# Autodesk Inventor assembly: am 42 Tooth Pulley Full
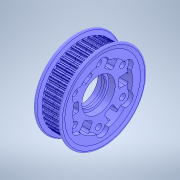
[picture p0: Inventor's stored thumbnail of the model, 180x180]
Saved by Autodesk Inventor 2021 (Build 250183000, 183)
## iProperties
Created: 2021-02-24
Part Number: am 42 Tooth Pulley Full
Document SubType Name: Assembly
Designer: aidan
Author: aidan
## Documents named in this file (2)
- C:\Users\aidan\Desktop\T3 Robotics\CAD\Generic and Stock\am 42 Tooth Pulley Full.iam
- C:\Users\aidan\Desktop\T3 Robotics\CAD\Generic and Stock\am 42 Tooth Pulley half.ipt
## Components (2 placed, 1 different names)
1. am 42 Tooth Pulley half:1 — Mate:2, Mate:3, Mate:4
2. am 42 Tooth Pulley half:2 — Mate:2, Mate:3, Mate:4
## Relationships (3: Mate 3)
- Mate:2: am 42 Tooth Pulley half:1 ↔ am 42 Tooth Pulley half:2
- Mate:3: am 42 Tooth Pulley half:1 ↔ am 42 Tooth Pulley half:2
- Mate:4: am 42 Tooth Pulley half:1 ↔ am 42 Tooth Pulley half:2
